# Autodesk Inventor assembly: PBT10
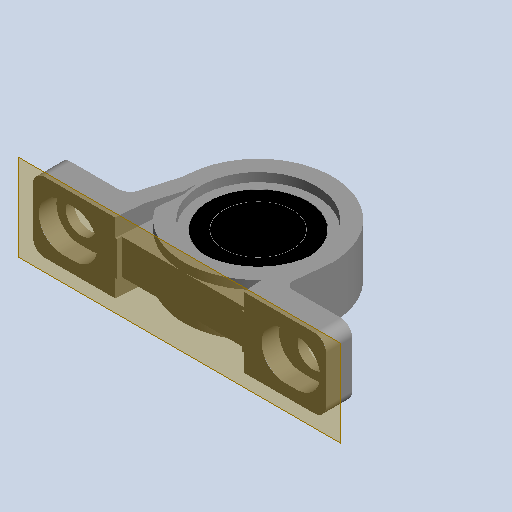
[picture p0: Inventor's stored thumbnail of the model, 512x512]
Saved by Autodesk Inventor 2023 (Build 270158000, 158)
## iProperties
Category: PARTsolutions
Company: MISUMI
Part Number: PBT10
Catalog Web Link: www.cadenas.de
Description: PBT, PBR, PBRS, PBRSX-Ball Bearing Units - Pillow Type
Vendor: MISUMI
Document SubType Name: Assembly
Designer: partserver
Manufacturer: MISUMI
Mass: 12.7142 g
Surface Area: 67.2375 cm^2
Volume: 12.7142 cm^3
Density: 1 g/cm^3
PSOL_IDENT_0: {$CADENAS_DATA\23d-libs\misumi\metric\12_bearing_holders\pbt_asmtab.prj},185 {VTYP=3D},{STYP=ASSTAB}
PSOL_IDENT_1: ,{NB=PBT10},{LINA=PBT10},{NN=PBT, PBR, PBRS, PBRSX},{DATE=18.06.2021 04:57:20},{GEOMDATE=08.06.2021
PSOL_IDENT_2: 06:41:11},{VERSION=},{LINEID=10},{WBVAR=TS,MAT},{WBNUMERIC=}  {NB=PBT10},{LINA=PBT10},{KT=DUMMY},{PN=
PSOL_IDENT_3: PBT10},{TYPE=PBT},{TS=T},{MAT=},{MATH=Zinc Alloy Die Cast},{MATB=52100 Bearing Steel},{MATRS=Nitrile
PSOL_IDENT_4: Rubber (NBR)},{MATSS=4137 Alloy Steel},{MATER=-},{STER=-},{PRECISION=JIS B 1558/JIS B 1559},{OT=-10
PSOL_IDENT_5: ~+ 80},{D=10},{H=18},{L=67},{L1=53},{A=16},{DD=7},{TT=6},{TX1=6},{TX2=5},{H1=35.0},{H11=35},{H12=34
PSOL_IDENT_6: .0},{B=14.0},{B1=17.500},{B2=14.000},{S=4.0},{MASS=70},{CR=4600},{CR1=4600},{CR2=3900},{COR=2000},{C
PSOL_IDENT_7: OR1=2000},{COR2=1550},{W1=70},{W2=77},{W3=79},{D1=17.000},{D2=12.000},{D3=34.000},{D4=36.000},{D5=26
PSOL_IDENT_8: .500},{M1=M3 x 0.35},{M2=M4 x 0.7},{TT1=0.59},{TT2=1.5},{ALC1=0.35},{ALC2=0.88},{MMIN1=2.621},{MMIN2=
PSOL_IDENT_9: 3.242},{MMAX1=3.000},{MMAX2=4.000},{M=M3 x 0.35},{T=0.59},{ALC=0.35},{MMIN=2.621},{MMAX=3},{MATALG=
PSOL_IDENT_10: '','Steel'     },{X=1},{DSCREW=3},{LSCREW=4},{DS1=3.000},{LS1=4.000},{DS2=4.000},{LS2=4.000},{D6=
PSOL_IDENT_11: 3.500},{PPATH=pbt_asmtpl.prj}
NB: PBT10
NN: PBT, PBR, PBRS, PBRSX
NT: Ball Bearing Units - Pillow Type
NBSYN: $PN.
LINA: PBT10
CATALOG: Misumi
TYPE: PBT
TS: Set Screw
MAT: Steel
MATH: Zinc Alloy Die Cast
MATB: 52100 Bearing Steel
MATRS: Nitrile Rubber (NBR)
MATSS: 4137 Alloy Steel
MATER: -
STER: -
PRECISION: JIS B 1558/JIS B 1559
OT: -10 ~+ 80
D: 10
H: 18
L: 67
L1: 53
A: 16
DD: 7
TT: 6
H1: 35
B: 14
S: 4
MASS: 70
CR: 4600
COR: 2000
M: M3 x 0.35
T: 0.59
ALC: 0.35
SUPPLIER: MISUMI
ARTICLENO: PBT10
BOMINFO: PBT10
CREATOR: CADENAS GmbH
Title: PBT10
Author: Cadenas PARTsolutions
Comments: Ball Bearing Units - Pillow Type
## Documents named in this file (3)
- C:\Users\田之上巧太\Documents\Basic_Parts\BasicParts\Bearing\PBT10\PBT10.iam
- C:\Users\田之上巧太\Documents\Basic_Parts\BasicParts\Bearing\PBT10\PBT10x.ipt
- C:\Users\田之上巧太\Documents\Basic_Parts\BasicParts\Bearing\PBT10\Hexagon socket set screw with flat point DIN 913 - M3x4.ipt
## Components (3 placed, 2 different names)
1. PBT10x:1 — to_screw_XY@1 <-> IP2_XY@2, to_screw_Z@1 <-> IP2_Z@2, to_screw_YZ@1 <-> IP2_YZ@2, to_screw_s_XY@1 <-> IP2_XY@3, to_screw_s_Z@1 <-> IP2_Z@3, to_screw_s_YZ@1 <-> IP2_YZ@3, メイト:5, 角度:3
2. Hexagon socket set screw with flat point DIN 913 - M3x4:1 — to_screw_XY@1 <-> IP2_XY@2, to_screw_Z@1 <-> IP2_Z@2, to_screw_YZ@1 <-> IP2_YZ@2
3. Hexagon socket set screw with flat point DIN 913 - M3x4:2 — to_screw_s_XY@1 <-> IP2_XY@3, to_screw_s_Z@1 <-> IP2_Z@3, to_screw_s_YZ@1 <-> IP2_YZ@3
## Relationships (8: Mate 5, Angle 3)
- to_screw_XY@1 <-> IP2_XY@2 [Mate]: PBT10x:1 ↔ Hexagon socket set screw with flat point DIN 913 - M3x4:1
- to_screw_Z@1 <-> IP2_Z@2 [Mate]: PBT10x:1 ↔ Hexagon socket set screw with flat point DIN 913 - M3x4:1
- to_screw_YZ@1 <-> IP2_YZ@2 [Angle] (0 deg): PBT10x:1 ↔ Hexagon socket set screw with flat point DIN 913 - M3x4:1
- to_screw_s_XY@1 <-> IP2_XY@3 [Mate]: PBT10x:1 ↔ Hexagon socket set screw with flat point DIN 913 - M3x4:2
- to_screw_s_Z@1 <-> IP2_Z@3 [Mate]: PBT10x:1 ↔ Hexagon socket set screw with flat point DIN 913 - M3x4:2
- to_screw_s_YZ@1 <-> IP2_YZ@3 [Angle] (0 deg): PBT10x:1 ↔ Hexagon socket set screw with flat point DIN 913 - M3x4:2
- メイト:5 [Mate]: PBT10x:1
- 角度:3 [Angle] (0 deg): PBT10x:1
